# Autodesk Inventor assembly: Fully Constrained 2 Speed Ball Shifter
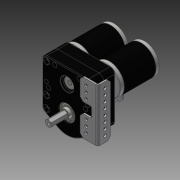
[picture p0: Inventor's stored thumbnail of the model, 180x180]
Saved by Autodesk Inventor 2014 SP1 (Build 180222100, 222)
## iProperties
Created: 2014-01-07
Part Number: Fully Constrained 2 Speed Ball Shifter
Document SubType Name: Assembly
Designer: Andrew Toennies
Mass: 3039.07 g
Surface Area: 3238.23 cm^2
Volume: 929.907 cm^3
Density: 3.26814 g/cm^3
Title: 217-2428 wUS Digital Encoder.20130115.STEP
Description: STEP AP203
Creation Date: 2013-01-14
Sending System: SolidWorks 2012
Preprocessor: SwSTEP 2.0
Author: Andrew Toennies
## Documents named in this file (32)
- C:\Users\Moses\Documents\Inventor\Robot\Constrained 2 Speed Ball Shifter\Fully Constrained 2 Speed Ball Shifter.iam
- C:\Users\Moses\Documents\Inventor\Robot\Constrained 2 Speed Ball Shifter\217-2733.ipt
- C:\Users\Moses\Documents\Inventor\Robot\Constrained 2 Speed Ball Shifter\217-2731.ipt
- C:\Users\Moses\Documents\Inventor\Robot\Constrained 2 Speed Ball Shifter\217-2789.ipt
- C:\Users\Moses\Documents\Inventor\Robot\Constrained 2 Speed Ball Shifter\217-2778-001 Rev2_NCQ8A075-050M.iam
- C:\Users\Moses\Documents\Inventor\Robot\Constrained 2 Speed Ball Shifter\217-2428-027 Rev1_97414A630.ipt
- C:\Users\Moses\Documents\Inventor\Robot\Constrained 2 Speed Ball Shifter\217-2788_57155K375.ipt
- C:\Users\Moses\Documents\Inventor\Robot\Constrained 2 Speed Ball Shifter\217-2428-012 Rev2.ipt
- C:\Users\Moses\Documents\Inventor\Robot\Constrained 2 Speed Ball Shifter\217-2428-005 Rev1.ipt
- C:\Users\Moses\Documents\Inventor\Robot\Constrained 2 Speed Ball Shifter\SCREW-832-0375.ipt
- C:\Users\Moses\Documents\Inventor\Robot\Constrained 2 Speed Ball Shifter\SBS1_SBS-0632-0250.ipt
- C:\Users\Moses\Documents\Inventor\Robot\Constrained 2 Speed Ball Shifter\217-2428-031 Rev1.iam
- C:\Users\Moses\Documents\Inventor\Robot\Constrained 2 Speed Ball Shifter\217-2428-016 Rev2_Spur01.ipt
- C:\Users\Moses\Documents\Inventor\Robot\Constrained 2 Speed Ball Shifter\217-2428-018 Rev2.ipt
- C:\Users\Moses\Documents\Inventor\Robot\Constrained 2 Speed Ball Shifter\217-2428-009 Rev1.ipt
- C:\Users\Moses\Documents\Inventor\Robot\Constrained 2 Speed Ball Shifter\SCREW-832-0250.ipt
- C:\Users\Moses\Documents\Inventor\Robot\Constrained 2 Speed Ball Shifter\217-2428-024 Rev2.ipt
- C:\Users\Moses\Documents\Inventor\Robot\Constrained 2 Speed Ball Shifter\SBS1_SBS1032-0500ZC.ipt
- C:\Users\Moses\Documents\Inventor\Robot\Constrained 2 Speed Ball Shifter\217-2614-001_12t.ipt
- C:\Users\Moses\Documents\Inventor\Robot\Constrained 2 Speed Ball Shifter\217-2761-001 rev1.ipt
- C:\Users\Moses\Documents\Inventor\Robot\Constrained 2 Speed Ball Shifter\217-2428-001 Rev1.ipt
- C:\Users\Moses\Documents\Inventor\Robot\Constrained 2 Speed Ball Shifter\217-2428-002 Rev2.ipt
- C:\Users\Moses\Documents\Inventor\Robot\Constrained 2 Speed Ball Shifter\217-2703-001.ipt
- C:\Users\Moses\Documents\Inventor\Robot\Constrained 2 Speed Ball Shifter\217-2707-001_40t.ipt
- C:\Users\Moses\Documents\Inventor\Robot\Constrained 2 Speed Ball Shifter\Nylock Nut_NNY2520-ZC.ipt
- C:\Users\Moses\Documents\Inventor\Robot\Constrained 2 Speed Ball Shifter\217-2428-004 Rev3.ipt
- C:\Users\Moses\Documents\Inventor\Robot\Constrained 2 Speed Ball Shifter\217-2428-021 Rev1.ipt
- C:\Users\Moses\Documents\Inventor\Robot\Constrained 2 Speed Ball Shifter\217-2428-029 Rev1.ipt
- C:\Users\Moses\Documents\Inventor\Robot\Constrained 2 Speed Ball Shifter\217-2792-001 Rev1.iam
- C:\Users\Moses\Documents\Inventor\Robot\Constrained 2 Speed Ball Shifter\E4P-X-250-X-D-D-D-X.ipt
- C:\Users\Moses\Documents\Inventor\Robot\Constrained 2 Speed Ball Shifter\217-2428-200 Rev1.iam
- C:\Users\Moses\Documents\Inventor\Robot\Constrained 2 Speed Ball Shifter\minicim.ipt
## Components (49 placed, 48 different names)
1. 217-2733_1 — Mate:12, Insert:20
2. 217-2733_2 — Mate:11, Insert:18, Insert:19
3. 217-2731_3 — Insert:22, Mate:19, Mate:20
4. 217-2789_4 — Insert:21
5. 217-2778-001 Rev2_NCQ8A075-050M_5 [sub-assembly] — Mate:8, Mate:9, Angle:1, Mate:26
6. 217-2428-027 Rev1_97414A630_6
7. 217-2788_57155K375_7
8. 217-2428-012 Rev2_8 — Insert:3, Mate:7, Insert:4, Insert:5, Mate:9, Angle:1, Insert:12, Insert:13, Mate:25, Mate:26
9. 217-2428-027 Rev1_97414A630_9
10. 217-2428-005 Rev1_10 — Insert:2, Insert:3
11. 217-2428-005 Rev1_11 — Insert:1, Mate:7
12. SCREW-832-0375_12 — Insert:5
13. SCREW-832-0375_13 — Insert:4
14. SCREW-832-0375_14 — Insert:9
15. SCREW-832-0375_15 — Insert:8
16. SBS1_SBS-0632-0250_16 — Insert:12
17. SBS1_SBS-0632-0250_17 — Insert:13
18. 217-2428-031 Rev1_18 [sub-assembly] — Mate:14, Flush:1, Rotation:6
19. 217-2428-016 Rev2_Spur01_19 — Mate:18, Mate:19, Rotation:5, Rotation:6
20. 217-2428-018 Rev2_20 — Insert:6, Insert:7, Mate:14, Flush:1, Mate:15, Mate:16, Mate:17, Insert:28, Mate:24
21. 217-2428-009 Rev1_21 — Insert:24, Mate:17
22. 217-2428-009 Rev1_22 — Insert:23, Mate:15, Mate:16
23. SCREW-832-0250_23 — Insert:7
24. SCREW-832-0375_24 — Insert:10
25. SCREW-832-0375_25 — Insert:11
26. SCREW-832-0250_26 — Insert:6
27. 217-2428-024 Rev2_27 — Mate:21, Mate:22, Mate:23
28. SBS1_SBS1032-0500ZC_28 — Mate:1, Insert:16
29. SBS1_SBS1032-0500ZC_29 — Mate:2, Insert:17
30. 217-2614-001_12t_30 — Insert:29, Rotation:3
31. 217-2761-001 rev1_31
32. SBS1_SBS1032-0500ZC_32 — Mate:5, Insert:14
33. SBS1_SBS1032-0500ZC_33 — Mate:4, Insert:15
34. 217-2761-001 rev1_34
35. 217-2614-001_12t_35 — Insert:30, Rotation:4
36. 217-2428-001 Rev1_36 — Mate:3, Mate:6, Insert:1, Insert:2, Insert:8, Insert:9, Insert:10, Insert:11, Insert:14, Insert:15, Insert:16, Insert:17, Insert:19, Insert:22, Insert:23, Insert:24, Mate:18
37. Nylock Nut_NNY2520-ZC_40
38. 217-2428-002 Rev2_37 — Insert:20, Insert:21, Mate:21, Mate:22, Mate:23
39. 217-2703-001_38 — Insert:27, Angle:4, Rotation:1
40. 217-2707-001_40t_39 — Insert:26, Angle:3, Insert:27, Flush:2, Rotation:2, Rotation:3, Rotation:4
41. Nylock Nut_NNY2520-ZC_41
42. 217-2428-004 Rev3_42 — Insert:18, Mate:13, Mate:10, Angle:3, Angle:4
43. 217-2428-021 Rev1_43 — Mate:10, Mate:11, Insert:26
44. 217-2428-029 Rev1_44 — Mate:12, Mate:13
45. 217-2792-001 Rev1_45 [sub-assembly] — Flush:2, Mate:20, Rotation:1, Rotation:2, Rotation:5, Rotation:7
46. E4P-X-250-X-D-D-D-X_48 — Insert:28, Mate:24
47. 217-2428-200 Rev1_49 [sub-assembly] — Mate:8, Rotation:7, Mate:25
48. minicim:1 — Mate:4, Mate:5, Mate:6, Insert:30
49. minicim:2 — Mate:1, Mate:2, Mate:3, Insert:29
## Relationships (67: Insert 29, Mate 26, RelateRotation 7, Angle 3, Flush 2)
- Mate:1: SBS1_SBS1032-0500ZC_28 ↔ minicim:2
- Mate:2: SBS1_SBS1032-0500ZC_29 ↔ minicim:2
- Mate:3: 217-2428-001 Rev1_36 ↔ minicim:2
- Mate:4: SBS1_SBS1032-0500ZC_33 ↔ minicim:1
- Mate:5: SBS1_SBS1032-0500ZC_32 ↔ minicim:1
- Mate:6: 217-2428-001 Rev1_36 ↔ minicim:1
- Insert:1: 217-2428-005 Rev1_11 ↔ 217-2428-001 Rev1_36
- Insert:2: 217-2428-005 Rev1_10 ↔ 217-2428-001 Rev1_36
- Insert:3: 217-2428-012 Rev2_8 ↔ 217-2428-005 Rev1_10
- Mate:7: 217-2428-012 Rev2_8 ↔ 217-2428-005 Rev1_11
- Insert:4: 217-2428-012 Rev2_8 ↔ SCREW-832-0375_13
- Insert:5: 217-2428-012 Rev2_8 ↔ SCREW-832-0375_12
- Insert:6: 217-2428-018 Rev2_20 ↔ SCREW-832-0250_26
- Insert:7: 217-2428-018 Rev2_20 ↔ SCREW-832-0250_23
- Insert:8: SCREW-832-0375_15 ↔ 217-2428-001 Rev1_36
- Insert:9: SCREW-832-0375_14 ↔ 217-2428-001 Rev1_36
- Insert:10: SCREW-832-0375_24 ↔ 217-2428-001 Rev1_36
- Insert:11: SCREW-832-0375_25 ↔ 217-2428-001 Rev1_36
- Mate:8: 217-2778-001 Rev2_NCQ8A075-050M_5 ↔ 217-2428-200 Rev1_49
- Mate:9: 217-2778-001 Rev2_NCQ8A075-050M_5 ↔ 217-2428-012 Rev2_8
- Angle:1 (0 deg): 217-2778-001 Rev2_NCQ8A075-050M_5 ↔ 217-2428-012 Rev2_8
- Insert:12: 217-2428-012 Rev2_8 ↔ SBS1_SBS-0632-0250_16
- Insert:13: 217-2428-012 Rev2_8 ↔ SBS1_SBS-0632-0250_17
- Insert:14: SBS1_SBS1032-0500ZC_32 ↔ 217-2428-001 Rev1_36
- Insert:15: SBS1_SBS1032-0500ZC_33 ↔ 217-2428-001 Rev1_36
- Insert:16: SBS1_SBS1032-0500ZC_28 ↔ 217-2428-001 Rev1_36
- Insert:17: SBS1_SBS1032-0500ZC_29 ↔ 217-2428-001 Rev1_36
- Mate:10: 217-2428-004 Rev3_42 ↔ 217-2428-021 Rev1_43
- Mate:11: 217-2733_2 ↔ 217-2428-021 Rev1_43
- Insert:18: 217-2733_2 ↔ 217-2428-004 Rev3_42
- Insert:19: 217-2733_2 ↔ 217-2428-001 Rev1_36
- Mate:12: 217-2733_1 ↔ 217-2428-029 Rev1_44
- Mate:13: 217-2428-004 Rev3_42 ↔ 217-2428-029 Rev1_44
- Insert:20: 217-2733_1 ↔ 217-2428-002 Rev2_37
- Insert:21: 217-2789_4 ↔ 217-2428-002 Rev2_37
- Insert:22: 217-2731_3 ↔ 217-2428-001 Rev1_36
- Mate:14: 217-2428-031 Rev1_18 ↔ 217-2428-018 Rev2_20
- Flush:1 (-10.3505 mm): 217-2428-031 Rev1_18 ↔ 217-2428-018 Rev2_20
- Insert:23: 217-2428-009 Rev1_22 ↔ 217-2428-001 Rev1_36
- Insert:24: 217-2428-009 Rev1_21 ↔ 217-2428-001 Rev1_36
- Mate:15: 217-2428-018 Rev2_20 ↔ 217-2428-009 Rev1_22
- Mate:16: 217-2428-018 Rev2_20 ↔ 217-2428-009 Rev1_22
- Mate:17: 217-2428-018 Rev2_20 ↔ 217-2428-009 Rev1_21
- Mate:18 (0.4767 mm): 217-2428-016 Rev2_Spur01_19 ↔ 217-2428-001 Rev1_36
- Mate:19: 217-2731_3 ↔ 217-2428-016 Rev2_Spur01_19
- Insert:26 (0.0254 mm): 217-2707-001_40t_39 ↔ 217-2428-021 Rev1_43
- Angle:3 (0 deg): 217-2707-001_40t_39 ↔ 217-2428-004 Rev3_42
- Insert:27 (0.0508 mm): 217-2703-001_38 ↔ 217-2707-001_40t_39
- Angle:4 (0 deg): 217-2703-001_38 ↔ 217-2428-004 Rev3_42
- Flush:2: 217-2707-001_40t_39 ↔ 217-2792-001 Rev1_45
- Mate:20: 217-2731_3 ↔ 217-2792-001 Rev1_45
- Rotation:1 [RelateRotation] (0.4 ul): 217-2703-001_38 ↔ 217-2792-001 Rev1_45
- Rotation:2 [RelateRotation] (0.9091 ul): 217-2707-001_40t_39 ↔ 217-2792-001 Rev1_45
- Mate:21: 217-2428-024 Rev2_27 ↔ 217-2428-002 Rev2_37
- Mate:22: 217-2428-024 Rev2_27 ↔ 217-2428-002 Rev2_37
- Mate:23: 217-2428-024 Rev2_27 ↔ 217-2428-002 Rev2_37
- Insert:28: 217-2428-018 Rev2_20 ↔ E4P-X-250-X-D-D-D-X_48
- Mate:24: 217-2428-018 Rev2_20 ↔ E4P-X-250-X-D-D-D-X_48
- Insert:29 (4.594 mm): 217-2614-001_12t_30 ↔ minicim:2
- Insert:30 (4.594 mm): 217-2614-001_12t_35 ↔ minicim:1
- Rotation:3 [RelateRotation] (0.3 ul): 217-2614-001_12t_30 ↔ 217-2707-001_40t_39
- Rotation:4 [RelateRotation] (0.3 ul): 217-2614-001_12t_35 ↔ 217-2707-001_40t_39
- Rotation:5 [RelateRotation] (1 ul): 217-2428-016 Rev2_Spur01_19 ↔ 217-2792-001 Rev1_45
- Rotation:6 [RelateRotation] (3 ul): 217-2428-031 Rev1_18 ↔ 217-2428-016 Rev2_Spur01_19
- Rotation:7 [RelateRotation] (1 ul): 217-2792-001 Rev1_45 ↔ 217-2428-200 Rev1_49
- Mate:25 (1.016 mm): 217-2428-012 Rev2_8 ↔ 217-2428-200 Rev1_49
- Mate:26: 217-2778-001 Rev2_NCQ8A075-050M_5 ↔ 217-2428-012 Rev2_8
